# Autodesk Inventor assembly: 01_Laser_Assy
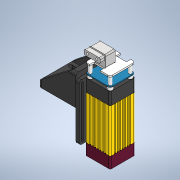
[picture p0: Inventor's stored thumbnail of the model, 180x180]
Saved by Autodesk Inventor 2022 (Build 260153000, 153)
## iProperties
Created: 2022-05-03
Part Number: 01_Laser_Assy
Document SubType Name: Assembly
Designer: MXBD
Author: MXBD
## Documents named in this file (8)
- A:\02_Laser_Engraver\CAD\Assembly\01_Laser_Assy.iam
- A:\02_Laser_Engraver\CAD\Parts\26_Laser_carriage_V2.ipt
- A:\02_Laser_Engraver\CAD\Parts\24_Laserholder.ipt
- A:\02_Laser_Engraver\CAD\Parts\13_Lasermodule_10W.ipt
- C:\Users\49152\Documents\Inventor\Content Center Files\R2022\de-DE\ISO 4762(2)\ISO 4762 - M3 x 6ISO.ipt
- C:\Users\49152\Documents\Inventor\Content Center Files\R2022\de-DE\ISO 4762(2)\ISO 4762 - M3 x 10ISO.ipt
- A:\02_Laser_Engraver\CAD\Parts\29_Lasercable_holder_A.ipt
- A:\02_Laser_Engraver\CAD\Parts\30_Lasercable_holder_B.ipt
## Components (11 placed, 7 different names)
1. 26_Laser_carriage_V2:1 — Passend:8, Passend:9, Passend:10, Passend:11, Passend:12, Passend:13
2. 24_Laserholder:1 — Passend:1, Passend:2, Passend:3, Passend:4, Passend:5, Passend:6, Passend:7, Passend:8, Passend:9, Passend:14, Passend:15, Passend:16, Passend:17
3. 13_Lasermodule_10W:1 — Passend:1, Passend:2, Passend:3, Mate:18, Flush:1, Flush:2
4. ISO 4762 M3 x 6:1 — Passend:4, Passend:7
5. ISO 4762 M3 x 6:2 — Passend:5, Passend:6
6. ISO 4762 M3 x 10:1 — Passend:11, Passend:14
7. ISO 4762 M3 x 10:2 — Passend:13, Passend:16
8. ISO 4762 M3 x 10:3 — Passend:12, Passend:17
9. ISO 4762 M3 x 10:4 — Passend:10, Passend:15
10. 29_Lasercable_holder_A:1 — Mate:18, Flush:1, Flush:2, Mate:19, Mate:20, Mate:21
11. 30_Lasercable_holder_B:1 — Mate:19, Mate:20, Mate:21
## Relationships (23: Mate 21, Flush 2)
- Passend:1 [Mate]: 24_Laserholder:1 ↔ 13_Lasermodule_10W:1
- Passend:2 [Mate]: 24_Laserholder:1 ↔ 13_Lasermodule_10W:1
- Passend:3 [Mate]: 24_Laserholder:1 ↔ 13_Lasermodule_10W:1
- Passend:4 [Mate]: 24_Laserholder:1 ↔ ISO 4762 M3 x 6:1
- Passend:5 [Mate]: 24_Laserholder:1 ↔ ISO 4762 M3 x 6:2
- Passend:6 [Mate]: 24_Laserholder:1 ↔ ISO 4762 M3 x 6:2
- Passend:7 [Mate]: 24_Laserholder:1 ↔ ISO 4762 M3 x 6:1
- Passend:8 [Mate]: 26_Laser_carriage_V2:1 ↔ 24_Laserholder:1
- Passend:9 [Mate]: 26_Laser_carriage_V2:1 ↔ 24_Laserholder:1
- Passend:10 [Mate]: 26_Laser_carriage_V2:1 ↔ ISO 4762 M3 x 10:4
- Passend:11 [Mate]: 26_Laser_carriage_V2:1 ↔ ISO 4762 M3 x 10:1
- Passend:12 [Mate]: 26_Laser_carriage_V2:1 ↔ ISO 4762 M3 x 10:3
- Passend:13 [Mate]: 26_Laser_carriage_V2:1 ↔ ISO 4762 M3 x 10:2
- Passend:14 [Mate]: 24_Laserholder:1 ↔ ISO 4762 M3 x 10:1
- Passend:15 [Mate]: 24_Laserholder:1 ↔ ISO 4762 M3 x 10:4
- Passend:16 [Mate]: 24_Laserholder:1 ↔ ISO 4762 M3 x 10:2
- Passend:17 [Mate]: 24_Laserholder:1 ↔ ISO 4762 M3 x 10:3
- Mate:18: 13_Lasermodule_10W:1 ↔ 29_Lasercable_holder_A:1
- Flush:1: 13_Lasermodule_10W:1 ↔ 29_Lasercable_holder_A:1
- Flush:2: 13_Lasermodule_10W:1 ↔ 29_Lasercable_holder_A:1
- Mate:19: 29_Lasercable_holder_A:1 ↔ 30_Lasercable_holder_B:1
- Mate:20: 29_Lasercable_holder_A:1 ↔ 30_Lasercable_holder_B:1
- Mate:21 (2 mm): 29_Lasercable_holder_A:1 ↔ 30_Lasercable_holder_B:1
